# Autodesk Inventor assembly: insideHand
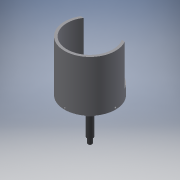
[picture p0: Inventor's stored thumbnail of the model, 180x180]
Saved by Autodesk Inventor 2016 (Build 200138000, 138)
## iProperties
Created: 2016-11-13
Part Number: insideHand
Material: 一般
Document SubType Name: Assembly
Designer: Daisuke
Author: Daisuke
## Documents named in this file (6)
- C:\Users\宏太\Documents\GitHub\CAD\Hand\ver2\insideHand.iam
- C:\Users\宏太\Documents\GitHub\CAD\Hand\ver2\Gear30.ipt
- C:\Users\宏太\Documents\GitHub\CAD\Hand\ver2\insideBottom1.ipt
- C:\Users\宏太\Documents\GitHub\CAD\Hand\ver2\InsideCover.ipt
- C:\Users\宏太\Documents\GitHub\CAD\Hand\ver2\STHRBN12_ss.ipt
- C:\Users\宏太\Documents\GitHub\CAD\Hand\ver2\SSFCU12-85-F12-P8.ipt
## Components (5 placed, 5 different names)
1. Gear30:1 — 挿入:4
2. insideBottom1:1 — 挿入:1, 挿入:2, 挿入:5, メイト:1
3. InsideCover:1 — 挿入:5, メイト:1
4. STHRBN12_ss:1 — 挿入:1, 挿入:2, 挿入:3, 挿入:4
5. SSFCU12-85-F12-P8:1 — 挿入:3
## Relationships (6: Insert 5, Mate 1)
- 挿入:1 [Insert]: insideBottom1:1 ↔ STHRBN12_ss:1
- 挿入:2 [Insert]: insideBottom1:1 ↔ STHRBN12_ss:1
- 挿入:3 [Insert]: STHRBN12_ss:1 ↔ SSFCU12-85-F12-P8:1
- 挿入:4 [Insert]: Gear30:1 ↔ STHRBN12_ss:1
- 挿入:5 [Insert]: insideBottom1:1 ↔ InsideCover:1
- メイト:1 [Mate]: insideBottom1:1 ↔ InsideCover:1
